# Autodesk Inventor assembly: Сборка2
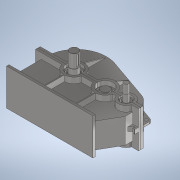
[picture p0: Inventor's stored thumbnail of the model, 180x180]
Saved by Autodesk Inventor 2022.1 (Build 261234020, 234B)
## iProperties
Created: 2021-12-09
Part Number: Сборка2
Document SubType Name: Assembly
Designer: Алексанян Г.
Author: Алексанян Г.
## Documents named in this file (6)
- C:\Users\Гарник\Desktop\учёба\5 семак\Детмаш\Reductor\Сборка2.iam
- C:\Users\Гарник\Desktop\учёба\5 семак\Детмаш\Reductor\МПСТ Корпус.ipt
- C:\Users\Гарник\Desktop\учёба\5 семак\Детмаш\Reductor\МПСТ Редуктор.iam
- C:\Users\Гарник\Desktop\учёба\5 семак\Детмаш\Reductor\МПСТ Крышка корпуса.ipt
- C:\Users\Гарник\Desktop\учёба\5 семак\Детмаш\Reductor\МПСТ Люк.ipt
- C:\Users\Гарник\Documents\Inventor\Content Center Files\R2022\ru-RU\End Cap GOST 13219·2-81\Крышка торцовая ГН 150 ГОСТ 13219.2-81.ipt
## Components (5 placed, 5 different names)
1. МПСТ Корпус:1 — Совмещение:1, Совмещение:2, Совмещение:3, Совмещение:4, Вставка:1, Совмещение:5, Вставка:2
2. МПСТ Редуктор:1 [sub-assembly] — Совмещение:1, Совмещение:2, Вставка:1
3. МПСТ Крышка корпуса:1 — Совмещение:3, Совмещение:4, Совмещение:5, Совмещение:6, Совмещение:7, Совмещение:8
4. МПСТ Люк:1 — Совмещение:6, Совмещение:7, Совмещение:8
5. Крышка торцовая ГОСТ 13219.2-81 ГН 150:1 — Вставка:2
## Relationships (10: Mate 8, Insert 2)
- Совмещение:1 [Mate]: МПСТ Корпус:1 ↔ МПСТ Редуктор:1
- Совмещение:2 [Mate]: МПСТ Корпус:1 ↔ МПСТ Редуктор:1
- Совмещение:3 [Mate]: МПСТ Корпус:1 ↔ МПСТ Крышка корпуса:1
- Совмещение:4 [Mate]: МПСТ Корпус:1 ↔ МПСТ Крышка корпуса:1
- Вставка:1 [Insert]: МПСТ Корпус:1 ↔ МПСТ Редуктор:1
- Совмещение:5 [Mate]: МПСТ Корпус:1 ↔ МПСТ Крышка корпуса:1
- Совмещение:6 [Mate]: МПСТ Крышка корпуса:1 ↔ МПСТ Люк:1
- Совмещение:7 [Mate]: МПСТ Крышка корпуса:1 ↔ МПСТ Люк:1
- Совмещение:8 [Mate]: МПСТ Крышка корпуса:1 ↔ МПСТ Люк:1
- Вставка:2 [Insert]: МПСТ Корпус:1 ↔ Крышка торцовая ГОСТ 13219.2-81 ГН 150:1
